# Autodesk Inventor assembly: Assembly1
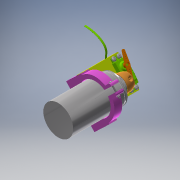
[picture p0: Inventor's stored thumbnail of the model, 180x180]
Saved by Autodesk Inventor 2016 (Build 200138000, 138)
## iProperties
Created: 2016-04-17
Part Number: Assembly1
Document SubType Name: Assembly
Designer: amenoni
Author: amenoni
## Documents named in this file (10)
- Z:\Desarrollo\WetMaths\wetMaths-Arduino\wetMaths\HwDesigns\Assembly1.iam
- Z:\Desarrollo\WetMaths\wetMaths-Arduino\wetMaths\HwDesigns\SprayCan.ipt
- Z:\Desarrollo\WetMaths\wetMaths-Arduino\wetMaths\HwDesigns\Clamp.ipt
- Z:\Desarrollo\WetMaths\wetMaths-Arduino\wetMaths\HwDesigns\CanNozzle.ipt
- Z:\Desarrollo\WetMaths\wetMaths-Arduino\wetMaths\HwDesigns\Futaba S3004.ipt
- Z:\Desarrollo\WetMaths\wetMaths-Arduino\wetMaths\HwDesigns\Servo_arm_np1.ipt
- Z:\Desarrollo\WetMaths\wetMaths-Arduino\wetMaths\HwDesigns\ServoSupport.ipt
- \\psf\Home\Documents\Inventor\Content Center Files\R2016\en-US\AS 1427(05)\AS 1427 - M2.5 x 25(5) II.ipt
- \\psf\Home\Documents\Inventor\Content Center Files\R2016\en-US\AS 1112 (2)\AS 1112 - M2.5  Type 5.ipt
- \\psf\Home\Documents\Inventor\Content Center Files\R2016\en-US\AS 1427(05)\AS 1427 - M4 x 6(5) II.ipt
## Components (12 placed, 9 different names)
1. SprayCan:1 — Mate:1, Mate:2, Mate:3
2. Clamp:1 — Mate:1, Mate:9, Mate:10, Mate:11, Insert:1, Insert:2
3. CanNozzle:1 — Mate:2, Mate:3
4. Futaba S3004:1 — Mate:4, Mate:5, Mate:6, Mate:7, Mate:8, Insert:3, Insert:4, Mate:12, Mate:13, Insert:5
5. Servo_arm_np1:1 — Mate:4, Mate:5
6. ServoSupport:1 — Mate:6, Mate:7, Mate:8, Mate:9, Mate:10, Mate:11
7. AS 1427 H - Metric M2.5 x 25:1 — Insert:1
8. AS 1112 (2) - Metric M2.5  Type 5:1 — Insert:2
9. AS 1427 H - Metric M4 x 6:1 — Insert:3
10. AS 1427 H - Metric M4 x 6:2 — Insert:4
11. AS 1427 H - Metric M4 x 6:3 — Mate:12, Mate:13
12. AS 1427 H - Metric M4 x 6:4 — Insert:5
## Relationships (18: Mate 13, Insert 5)
- Mate:1: SprayCan:1 ↔ Clamp:1
- Mate:2: SprayCan:1 ↔ CanNozzle:1
- Mate:3 (2.5 mm): SprayCan:1 ↔ CanNozzle:1
- Mate:4: Futaba S3004:1 ↔ Servo_arm_np1:1
- Mate:5: Futaba S3004:1 ↔ Servo_arm_np1:1
- Mate:6: Futaba S3004:1 ↔ ServoSupport:1
- Mate:7: Futaba S3004:1 ↔ ServoSupport:1
- Mate:8: Futaba S3004:1 ↔ ServoSupport:1
- Mate:9: Clamp:1 ↔ ServoSupport:1
- Mate:10: Clamp:1 ↔ ServoSupport:1
- Mate:11 (7 mm): Clamp:1 ↔ ServoSupport:1
- Insert:1: Clamp:1 ↔ AS 1427 H - Metric M2.5 x 25:1
- Insert:2: Clamp:1 ↔ AS 1112 (2) - Metric M2.5  Type 5:1
- Insert:3: Futaba S3004:1 ↔ AS 1427 H - Metric M4 x 6:1
- Insert:4: Futaba S3004:1 ↔ AS 1427 H - Metric M4 x 6:2
- Mate:12: Futaba S3004:1 ↔ AS 1427 H - Metric M4 x 6:3
- Mate:13: Futaba S3004:1 ↔ AS 1427 H - Metric M4 x 6:3
- Insert:5: Futaba S3004:1 ↔ AS 1427 H - Metric M4 x 6:4
